# Autodesk Inventor assembly: EsagonoScreeenChiuso
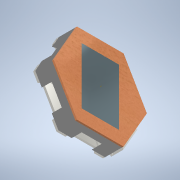
[picture p0: Inventor's stored thumbnail of the model, 180x180]
Saved by Autodesk Inventor 2020 (Build 240168000, 168)
## iProperties
Created: 2020-04-22
Part Number: EsagonoScreeenChiuso
Document SubType Name: Assembly
Designer: Samuele
Author: Samuele
## Documents named in this file (5)
- C:\EsagoniMalsani\ModelliComponenti\EsagonoScreeenChiuso.iam
- C:\EsagoniMalsani\ModelliComponenti\HexagoneBack.ipt
- C:\EsagoniMalsani\ModelliComponenti\TouchLCD.ipt
- C:\EsagoniMalsani\ModelliComponenti\FrontalinoWood.ipt
- C:\EsagoniMalsani\ModelliComponenti\HexagoneScreen.ipt
## Components (4 placed, 4 different names)
1. HexagoneBack:5 — Flush:1, Flush:2
2. TouchLCD:1
3. FrontalinoWood:1 — Mate:1
4. HexagoneScreen:1 — Flush:1, Flush:2, Mate:1
## Relationships (3: Flush 2, Mate 1)
- Flush:1: HexagoneBack:5 ↔ HexagoneScreen:1
- Flush:2: HexagoneBack:5 ↔ HexagoneScreen:1
- Mate:1: FrontalinoWood:1 ↔ HexagoneScreen:1
